# Autodesk Inventor assembly: cpu_module
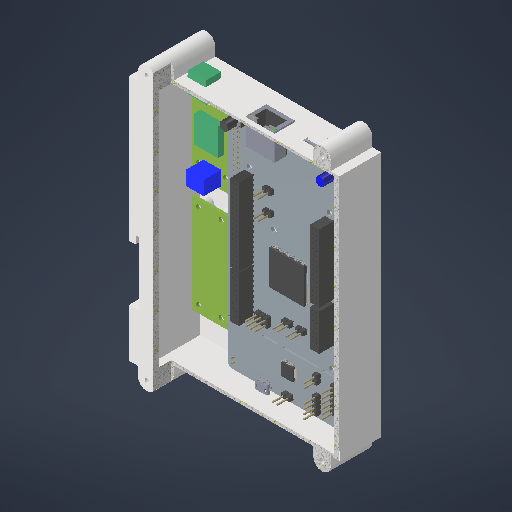
[picture p0: Inventor's stored thumbnail of the model, 512x512]
Saved by Autodesk Inventor 2025 (Build 290162000, 162)
## iProperties
Created: 2024-09-05
Part Number: cpu_module
Document SubType Name: Assembly
Designer: Dawid
Author: Dawid
## Documents named in this file (6)
- C:\Users\Dawid\Desktop\Magisterka\plc_io_module_case\cpu_module.iam
- C:\Users\Dawid\Desktop\Magisterka\plc_io_module_case\nucleo-f429zi-3d-model-step-56544-1.snapshot.1\NUCLEO-F429ZI--3DModel-STEP-56544.ipt
- C:\Users\Dawid\Desktop\Magisterka\plc_io_module_case\cpu_case.ipt
- cpu_case.ipt
- C:\Users\Dawid\Desktop\Magisterka\plc_io_module_case\buck_converter.ipt
- C:\Users\Dawid\Desktop\Magisterka\plc_io_module_case\bus_connector_board.ipt
## Components (4 placed, 4 different names)
1. NUCLEO-F429ZI--3DModel-STEP-56544:1
2. cpu_case:1
3. buck_converter:1
4. bus_connector_board:1
## Relationships (3: WeldJoint 3)
- [WeldJoint]: NUCLEO-F429ZI--3DModel-STEP-56544:1 ↔ cpu_case:1
- [WeldJoint]: cpu_case:1 ↔ buck_converter:1
- [WeldJoint]: cpu_case:1 ↔ bus_connector_board:1
